# Autodesk Inventor assembly: ASY ANP 1425 FDS way 5
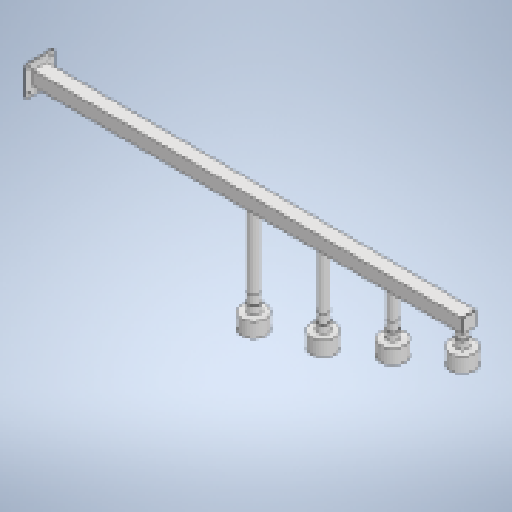
[picture p0: Inventor's stored thumbnail of the model, 512x512]
Saved by Autodesk Inventor 2025 (Build 290162010, 162A)
## iProperties
Created: 2025-07-02
Part Number: ASY ANP 1425 FDS way 5
Document SubType Name: Assembly
Designer: admin
Author: user
## Documents named in this file (9)
- C:\Users\pokla\Documents\Inventor\ANP--Antipayuta\FDS 1400\ASY ANP 1425 FDS way 5.iam
- C:\Users\pokla\Documents\Inventor\ANP--Antipayuta\FDS 1400\ANP 1435 FDS WAY tube5.ipt
- C:\Users\pokla\Documents\Inventor\ANP--Antipayuta\FDS 1400\ANP 1425 FDS Way FLANGE.ipt
- C:\Users\pokla\Documents\Inventor\ANP--Antipayuta\FDS 1400\ANP 1426 FDS way cup.ipt
- C:\Users\pokla\Documents\Inventor\ANP--Antipayuta\FDS 1400\ANP dummy filter element.ipt
- C:\Users\pokla\Documents\Inventor\ANP--Antipayuta\FDS 1400\ANP dummy pipe nippel.ipt
- C:\Users\pokla\Documents\Inventor\ANP--Antipayuta\FDS 1400\ANP 1448 FDS thread  tube8.ipt
- C:\Users\pokla\Documents\Inventor\ANP--Antipayuta\FDS 1400\ANP 1449 FDS thread  tube9.ipt
- C:\Users\pokla\Documents\Inventor\ANP--Antipayuta\FDS 1400\ANP 1451 FDS thread  tube10.ipt
## Components (14 placed, 8 different names)
1. ANP 1435 FDS WAY tube5.ipt:1 — Rigid:34, Rigid:35, Rigid:36, Rigid:53, Rigid:54, Rigid:55
2. ANP 1425 FDS Way FLANGE.ipt:1 — Rigid:34
3. ANP 1426 FDS way cup.ipt:1 — Rigid:35
4. ANP dummy filter element.ipt:1 — Rigid:1
5. ANP dummy pipe nippel.ipt:1 — Rigid:1, Rigid:44
6. ANP dummy filter element.ipt:2 — Rigid:6
7. ANP dummy pipe nippel.ipt:2 — Rigid:6, Rigid:46
8. ANP dummy filter element.ipt:4 — Rigid:14
9. ANP dummy pipe nippel.ipt:4 — Rigid:14, Rigid:45
10. ANP dummy filter element.ipt:6 — Rigid:33
11. ANP dummy pipe nippel.ipt:6 — Rigid:33, Rigid:36
12. ANP 1448 FDS thread  tube8.ipt:1 — Rigid:46, Rigid:53
13. ANP 1449 FDS thread  tube9.ipt:1 — Rigid:45, Rigid:54
14. ANP 1451 FDS thread  tube10.ipt:1 — Rigid:44, Rigid:55
## Relationships (13: WeldJoint 13)
- Rigid:34 [WeldJoint] (2 mm): ANP 1435 FDS WAY tube5.ipt:1 ↔ ANP 1425 FDS Way FLANGE.ipt:1
- Rigid:35 [WeldJoint]: ANP 1435 FDS WAY tube5.ipt:1 ↔ ANP 1426 FDS way cup.ipt:1
- Rigid:1 [WeldJoint]: ANP dummy filter element.ipt:1 ↔ ANP dummy pipe nippel.ipt:1
- Rigid:6 [WeldJoint]: ANP dummy filter element.ipt:2 ↔ ANP dummy pipe nippel.ipt:2
- Rigid:14 [WeldJoint]: ANP dummy filter element.ipt:4 ↔ ANP dummy pipe nippel.ipt:4
- Rigid:33 [WeldJoint]: ANP dummy filter element.ipt:6 ↔ ANP dummy pipe nippel.ipt:6
- Rigid:36 [WeldJoint]: ANP 1435 FDS WAY tube5.ipt:1 ↔ ANP dummy pipe nippel.ipt:6
- Rigid:46 [WeldJoint]: ANP dummy pipe nippel.ipt:2 ↔ ANP 1448 FDS thread  tube8.ipt:1
- Rigid:53 [WeldJoint]: ANP 1435 FDS WAY tube5.ipt:1 ↔ ANP 1448 FDS thread  tube8.ipt:1
- Rigid:45 [WeldJoint]: ANP dummy pipe nippel.ipt:4 ↔ ANP 1449 FDS thread  tube9.ipt:1
- Rigid:54 [WeldJoint]: ANP 1435 FDS WAY tube5.ipt:1 ↔ ANP 1449 FDS thread  tube9.ipt:1
- Rigid:44 [WeldJoint]: ANP dummy pipe nippel.ipt:1 ↔ ANP 1451 FDS thread  tube10.ipt:1
- Rigid:55 [WeldJoint]: ANP 1435 FDS WAY tube5.ipt:1 ↔ ANP 1451 FDS thread  tube10.ipt:1
